# Autodesk Inventor assembly: Test_zebatek_odl_rowna_srednicy
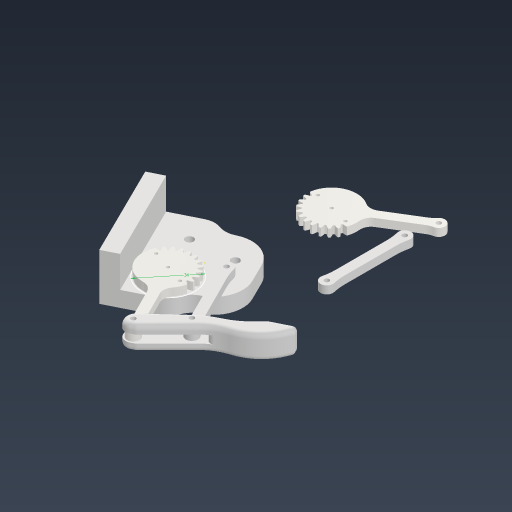
[picture p0: Inventor's stored thumbnail of the model, 512x512]
Saved by Autodesk Inventor 2024 (Build 280153000, 153)
## iProperties
Created: 2023-12-19
Part Number: Test_zebatek_odl_rowna_srednicy
Document SubType Name: Assembly
Designer: Piter
Author: Piter
## Documents named in this file (5)
- C:\Users\Piter\OneDrive\Pulpit\gripper\Mygripper\Test_zebatek_odl_rowna_srednicy.iam
- C:\Users\Piter\OneDrive\Pulpit\gripper\Mygripper\Zebatka_gut.ipt
- C:\Users\Piter\OneDrive\Pulpit\gripper\Mygripper\Podstawa.ipt
- C:\Users\Piter\OneDrive\Pulpit\gripper\Mygripper\Connector.ipt
- C:\Users\Piter\OneDrive\Pulpit\gripper\Mygripper\szczeka.ipt
## Components (6 placed, 4 different names)
1. Spur Gear2:1 — Rotational:2
2. Spur Gear2:2 — Rotational:1, Rotational:4, Mate:1, Mate:3, Rotational:5
3. Podstawa:1 — Rotational:1, Rotational:2, Rotational:3, Rotational:4
4. Connector:1 — Rotational:3, Mate:2, Mate:4
5. Connector:2
6. szczeka:1 — Mate:1, Mate:2, Mate:3, Rotational:5, Mate:4
## Relationships (9: RevoluteJoint 5, Mate 4)
- Rotational:1 [RevoluteJoint]: Spur Gear2:2 ↔ Podstawa:1
- Rotational:2 [RevoluteJoint]: Spur Gear2:1 ↔ Podstawa:1
- Rotational:3 [RevoluteJoint]: Podstawa:1 ↔ Connector:1
- Rotational:4 [RevoluteJoint]: Spur Gear2:2 ↔ Podstawa:1
- Mate:1: Spur Gear2:2 ↔ szczeka:1
- Mate:2: Connector:1 ↔ szczeka:1
- Mate:3: Spur Gear2:2 ↔ szczeka:1
- Rotational:5 [RevoluteJoint]: Spur Gear2:2 ↔ szczeka:1
- Mate:4: Connector:1 ↔ szczeka:1
